# Autodesk Inventor assembly: base long wall
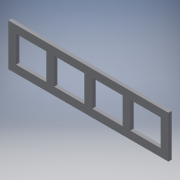
[picture p0: Inventor's stored thumbnail of the model, 180x180]
Saved by Autodesk Inventor 2017 (Build 210142000, 142)
## iProperties
Created: 2019-05-05
Part Number: base long wall
Document SubType Name: Assembly
Designer: Roman
Author: Roman
## Documents named in this file (3)
- C:\Users\Roman\Documents\CAD\tegu rev2\base\long wall\base long wall.iam
- C:\Users\Roman\Documents\CAD\tegu rev2\base\long wall\base long wall h bar.ipt
- C:\Users\Roman\Documents\CAD\tegu rev2\base\long wall\base long wall v bar.ipt
## Components (7 placed, 2 different names)
1. base long wall h bar:1 — Mate:1, Flush:1, Flush:2
2. base long wall h bar:2 — Mate:2, Flush:3, Flush:4
3. base long wall v bar:1 — Mate:1, Flush:1, Flush:2, Mate:2, Flush:3, Flush:4
4. base long wall v bar:2
5. base long wall v bar:3
6. base long wall v bar:4
7. base long wall v bar:5
## Component patterns: (5 elements, first: base long wall v bar:1)
## Relationships (6: Flush 4, Mate 2)
- Mate:1: base long wall h bar:1 ↔ base long wall v bar:1
- Flush:1: base long wall h bar:1 ↔ base long wall v bar:1
- Flush:2: base long wall h bar:1 ↔ base long wall v bar:1
- Mate:2: base long wall h bar:2 ↔ base long wall v bar:1
- Flush:3: base long wall h bar:2 ↔ base long wall v bar:1
- Flush:4: base long wall h bar:2 ↔ base long wall v bar:1
